# Autodesk Inventor assembly: Stanina
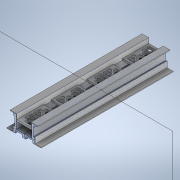
[picture p0: Inventor's stored thumbnail of the model, 180x180]
Saved by Autodesk Inventor 2022 (Build 260153000, 153)
## iProperties
Created: 2023-08-15
Part Number: Stanina
Document SubType Name: Assembly
Designer: Kippi
Author: Kippi
## Documents named in this file (5)
- C:\Users\Kippi\Documents\CNC_Lathe\Stanina.iam
- C:\Users\Kippi\Documents\CNC_Lathe\L_PlNKA800.ipt
- C:\Users\Kippi\Documents\CNC_Lathe\Ugol800.ipt
- C:\Users\Kippi\Documents\CNC_Lathe\L_PlNKA_Niz.ipt
- C:\Users\Kippi\Documents\CNC_Lathe\PlaskaUkrep.ipt
## Components (12 placed, 4 different names)
1. Ugol800:1 — Mate:10, Flush:11, Flush:12, Mate:14, Mate:15, Flush:16, Flush:17
2. Ugol800:2 — Mate:9, Mate:11, Flush:13, Mate:12, Mate:13, Flush:21, Mate:17, Mate:18
3. L_PlNKA_Niz:1 — Mate:1, Flush:1, Flush:2, Mate:8, Mate:16, Flush:18, Flush:19, Mate:20, Flush:25, Flush:27
4. L_PlNKA_Niz:2 — Mate:1, Flush:1, Flush:2, Mate:8, Mate:19, Flush:24, Flush:26
5. PlaskaUkrep:1 — Mate:9, Mate:10, Flush:11, Flush:12, Flush:23
6. PlaskaUkrep:2 — Mate:11, Flush:13, Flush:14, Flush:15, Flush:16, Flush:17, Flush:20, Flush:22
7. L_PlNKA800:3 — Mate:12, Mate:13, Flush:15, Flush:20, Flush:21
8. L_PlNKA800:4 — Mate:14, Mate:15, Flush:14, Mate:16, Flush:18, Flush:19
9. PlaskaUkrep:3 — Mate:17, Flush:22
10. PlaskaUkrep:4 — Flush:23, Mate:18
11. Ugol800:3 — Mate:20, Flush:25, Flush:27
12. Ugol800:4 — Mate:19, Flush:24, Flush:26
## Relationships (33: Flush 19, Mate 14)
- Mate:1: L_PlNKA_Niz:1 ↔ L_PlNKA_Niz:2
- Flush:1: L_PlNKA_Niz:1 ↔ L_PlNKA_Niz:2
- Flush:2: L_PlNKA_Niz:1 ↔ L_PlNKA_Niz:2
- Mate:8: L_PlNKA_Niz:1 ↔ L_PlNKA_Niz:2
- Mate:9: Ugol800:2 ↔ PlaskaUkrep:1
- Mate:10: Ugol800:1 ↔ PlaskaUkrep:1
- Flush:11: Ugol800:1 ↔ PlaskaUkrep:1
- Flush:12: Ugol800:1 ↔ PlaskaUkrep:1
- Mate:11: Ugol800:2 ↔ PlaskaUkrep:2
- Flush:13: Ugol800:2 ↔ PlaskaUkrep:2
- Mate:12: Ugol800:2 ↔ L_PlNKA800:3
- Mate:13: Ugol800:2 ↔ L_PlNKA800:3
- Mate:14: Ugol800:1 ↔ L_PlNKA800:4
- Mate:15: Ugol800:1 ↔ L_PlNKA800:4
- Flush:14: PlaskaUkrep:2 ↔ L_PlNKA800:4
- Flush:15: PlaskaUkrep:2 ↔ L_PlNKA800:3
- Flush:16: Ugol800:1 ↔ PlaskaUkrep:2
- Flush:17: Ugol800:1 ↔ PlaskaUkrep:2
- Mate:16: L_PlNKA_Niz:1 ↔ L_PlNKA800:4
- Flush:18: L_PlNKA_Niz:1 ↔ L_PlNKA800:4
- Flush:19: L_PlNKA_Niz:1 ↔ L_PlNKA800:4
- Flush:20: PlaskaUkrep:2 ↔ L_PlNKA800:3
- Flush:21: Ugol800:2 ↔ L_PlNKA800:3
- Mate:17: Ugol800:2 ↔ PlaskaUkrep:3
- Flush:22: PlaskaUkrep:2 ↔ PlaskaUkrep:3
- Flush:23: PlaskaUkrep:1 ↔ PlaskaUkrep:4
- Mate:18: Ugol800:2 ↔ PlaskaUkrep:4
- Mate:19: L_PlNKA_Niz:2 ↔ Ugol800:4
- Mate:20: L_PlNKA_Niz:1 ↔ Ugol800:3
- Flush:24: L_PlNKA_Niz:2 ↔ Ugol800:4
- Flush:25: L_PlNKA_Niz:1 ↔ Ugol800:3
- Flush:26: L_PlNKA_Niz:2 ↔ Ugol800:4
- Flush:27: L_PlNKA_Niz:1 ↔ Ugol800:3
